# Autodesk Inventor assembly: SklopReduktora
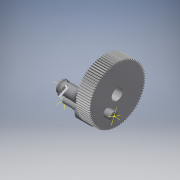
[picture p0: Inventor's stored thumbnail of the model, 180x180]
Saved by Autodesk Inventor 2018 (Build 220112000, 112)
## iProperties
Created: 2018-11-17
Part Number: SklopReduktora
Document SubType Name: Assembly
Designer: Kristijan
Author: Kristijan
## Documents named in this file (7)
- C:\Users\krist\Dropbox (Personal)\PolitehnikaPula\5 semestar\Konstrukcije\TimskiProjektniZadatak\OutputDrawings\SklopReduktora.iam
- C:\Users\krist\Dropbox (Personal)\PolitehnikaPula\5 semestar\Konstrukcije\TimskiProjektniZadatak\OutputDrawings\PogonskoVratilo.ipt
- C:\Users\krist\Dropbox (Personal)\PolitehnikaPula\5 semestar\Konstrukcije\TimskiProjektniZadatak\datasheetsModels\6008.iam
- C:\Users\krist\Dropbox (Personal)\PolitehnikaPula\5 semestar\Konstrukcije\TimskiProjektniZadatak\OutputDrawings\GonjenoVratilo.ipt
- C:\Users\krist\Dropbox (Personal)\PolitehnikaPula\5 semestar\Konstrukcije\TimskiProjektniZadatak\datasheetsModels\32913.iam
- C:\Users\krist\Dropbox (Personal)\PolitehnikaPula\5 semestar\Konstrukcije\TimskiProjektniZadatak\OutputDrawings\GonjeniZupcanik.ipt
- C:\Users\krist\Documents\Inventor\Content Center Files\R2018\en-US\DIN 6885-1 A\DIN 6885 - A 22 x 14 x 90.ipt
## Components (8 placed, 6 different names)
1. PogonskoVratilo:1 — Mate:1, Mate:3, Mate:4, Mate:5, Mate:10, Mate:12
2. 6008:1 [sub-assembly] — Mate:3, Mate:4
3. 6008:2 [sub-assembly] — Mate:1, Mate:5, Flush:14
4. GonjenoVratilo:1 — Mate:6, Mate:7, Mate:8, Mate:9, Mate:11
5. 32913:1 [sub-assembly] — Mate:6, Mate:7, Flush:14
6. 32913:2 [sub-assembly] — Mate:8, Mate:9
7. Spur Gear2:1
8. DIN 6885-1 A A 22 x 14 x 90:1
## Relationships (12: Mate 11, Flush 1)
- Mate:1: PogonskoVratilo:1 ↔ 6008:2
- Mate:3: PogonskoVratilo:1 ↔ 6008:1
- Mate:4: PogonskoVratilo:1 ↔ 6008:1
- Mate:5: PogonskoVratilo:1 ↔ 6008:2
- Mate:6: GonjenoVratilo:1 ↔ 32913:1
- Mate:7: GonjenoVratilo:1 ↔ 32913:1
- Mate:8: GonjenoVratilo:1 ↔ 32913:2
- Mate:9: GonjenoVratilo:1 ↔ 32913:2
- Mate:10: PogonskoVratilo:1
- Mate:11 (262.5 mm): GonjenoVratilo:1
- Mate:12: PogonskoVratilo:1
- Flush:14 (2.5 mm): 6008:2 ↔ 32913:1
